# Autodesk Inventor assembly: Papa John Test- Ty
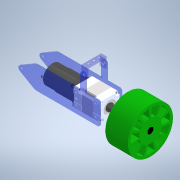
[picture p0: Inventor's stored thumbnail of the model, 180x180]
Saved by Autodesk Inventor 2020 (Build 240168000, 168)
## iProperties
Created: 2020-01-31
Part Number: Papa John Test- Ty
Document SubType Name: Assembly
Designer: aidan
Author: aidan
## Documents named in this file (7)
- C:\Users\aidan\Desktop\T3 Robotics\CAD\Papa John Test- Ty.iam
- C:\Users\aidan\Desktop\T3 Robotics\CAD\Papa John Bolt Plate.ipt
- C:\Users\aidan\Desktop\T3 Robotics\CAD\Papa John Mounting Plate.ipt
- C:\Users\aidan\Desktop\T3 Robotics\CAD\Generic and Stock\VersaPlanetary Parts\VersaPlanetary Two Stage 775.iam
- C:\Users\aidan\Desktop\T3 Robotics\CAD\Tony's CAD\Compliance wheel.ipt
- C:\Users\aidan\Desktop\T3 Robotics\CAD\Thundershaft 2in.ipt
- C:\Users\aidan\Desktop\T3 Robotics\CAD\Frame Test for Papa John.ipt
## Components (7 placed, 6 different names)
1. Papa John Bolt Plate:1 — Mate:1, Mate:2, Mate:10, Mate:11, Mate:12
2. Papa John Mounting Plate:1 — Mate:1, Mate:2, Mate:3, Mate:4, Mate:5
3. VersaPlanetary Two Stage 775:1 [sub-assembly] — Mate:3, Mate:4, Mate:5, Mate:7, Mate:8, Flush:9, Flush:10, Mate:9
4. Compliance wheel:1 — Flush:7, Flush:8, Mate:6, Mate:7, Mate:8, Flush:11
5. Compliance wheel:2 — Flush:7, Flush:8, Mate:6
6. Thundershaft 2in:1 — Flush:9, Flush:10, Mate:9, Flush:11
7. Frame Test for Papa John:1 — Mate:10, Mate:11, Mate:12
## Relationships (17: Mate 12, Flush 5)
- Mate:1: Papa John Bolt Plate:1 ↔ Papa John Mounting Plate:1
- Mate:2: Papa John Bolt Plate:1 ↔ Papa John Mounting Plate:1
- Mate:3: Papa John Mounting Plate:1 ↔ VersaPlanetary Two Stage 775:1
- Mate:4: Papa John Mounting Plate:1 ↔ VersaPlanetary Two Stage 775:1
- Mate:5: Papa John Mounting Plate:1 ↔ VersaPlanetary Two Stage 775:1
- Flush:7: Compliance wheel:1 ↔ Compliance wheel:2
- Flush:8: Compliance wheel:1 ↔ Compliance wheel:2
- Mate:6: Compliance wheel:1 ↔ Compliance wheel:2
- Mate:7: VersaPlanetary Two Stage 775:1 ↔ Compliance wheel:1
- Mate:8: VersaPlanetary Two Stage 775:1 ↔ Compliance wheel:1
- Flush:9: VersaPlanetary Two Stage 775:1 ↔ Thundershaft 2in:1
- Flush:10: VersaPlanetary Two Stage 775:1 ↔ Thundershaft 2in:1
- Mate:9: VersaPlanetary Two Stage 775:1 ↔ Thundershaft 2in:1
- Flush:11: Compliance wheel:1 ↔ Thundershaft 2in:1
- Mate:10: Papa John Bolt Plate:1 ↔ Frame Test for Papa John:1
- Mate:11: Papa John Bolt Plate:1 ↔ Frame Test for Papa John:1
- Mate:12: Papa John Bolt Plate:1 ↔ Frame Test for Papa John:1
